# Autodesk Inventor assembly: Assembly_Palu
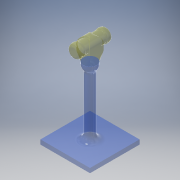
[picture p0: Inventor's stored thumbnail of the model, 180x180]
Saved by Autodesk Inventor 2017 (Build 210142000, 142)
## iProperties
Created: 2021-02-25
Part Number: Assembly_Palu
Document SubType Name: Assembly
Designer: Lenovo Y900
Author: Lenovo Y900
## Documents named in this file (3)
- D:\Sekolah\Skripsi\New Part\Assembly_Palu.iam
- D:\Sekolah\Skripsi\New Part\Base.ipt
- D:\Sekolah\Skripsi\New Part\Palu.ipt
## Components (2 placed, 2 different names)
1. Base:1 — Mate:1, Mate:2, Mate:3
2. Palu:1 — Mate:1, Mate:2, Mate:3
## Relationships (3: Mate 3)
- Mate:1: Base:1 ↔ Palu:1
- Mate:2: Base:1 ↔ Palu:1
- Mate:3: Base:1 ↔ Palu:1
